# Autodesk Inventor assembly: EC5 connector
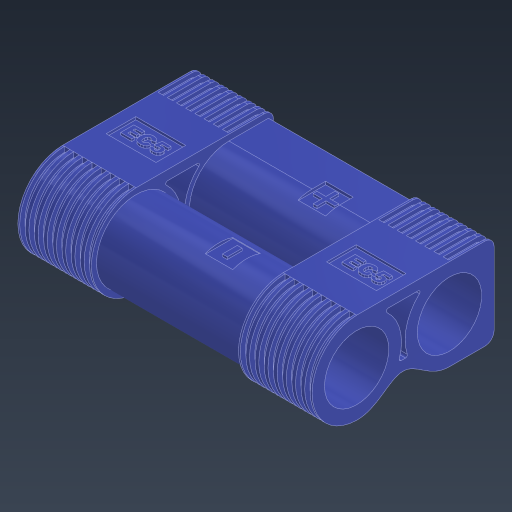
[picture p0: Inventor's stored thumbnail of the model, 512x512]
Saved by Autodesk Inventor 2023 (Build 270158000, 158)
## iProperties
Created: 2018-01-21
Part Number: EC5 connector
Document SubType Name: Assembly
Designer: szymo
Sending System: Autodesk Translation Framework v6.5.0.72
Preprocessor: ST-DEVELOPER v16.13
Title: /var/folders/jf/x3ls839j65x6dg684_w5j1x40000gn/T/com.autodesk.mas.fusion360/Neutron/9bf27b2e-ac52-47d8-a75e-b773bacf722d.stp
Author: glushkov.ag@me.com
## Documents named in this file (3)
- D:\tech\diy\e-skateboard\projekcik-inventor\EC5 connector v22.iam
- D:\tech\diy\e-skateboard\projekcik-inventor\BaseF.ipt
- D:\tech\diy\e-skateboard\projekcik-inventor\Base M.ipt
## Components (2 placed, 2 different names)
1. BaseF:1 — Mate:1, Flush:1, Flush:2
2. Base M:1 — Mate:1, Flush:1, Flush:2
## Relationships (3: Flush 2, Mate 1)
- Mate:1: BaseF:1 ↔ Base M:1
- Flush:1: BaseF:1 ↔ Base M:1
- Flush:2: BaseF:1 ↔ Base M:1
